# Autodesk Inventor assembly: Chargeur
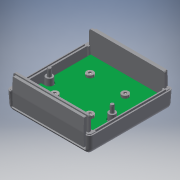
[picture p0: Inventor's stored thumbnail of the model, 180x180]
Saved by Autodesk Inventor 2016 SP1 (Build 200210100, 210)
## iProperties
Created: 2016-04-25
Part Number: Chargeur
Material: Générique
Document SubType Name: Assembly
Designer: dimercur
Sending System: Autodesk Inventor 2016
Preprocessor: unknown
Minimum Resolution: 0.01
Sent Units: Millimeter
Translation Standard: IGES 5.3
Model Creation Time: 2016-02-17
Title: 1593K.iam
Author: MBeerman
## Documents named in this file (8)
- D:\Users\dimercur\Documents\SVN\projets-gei\Dumber 2015\Mecanique\Chargeur\Chargeur.iam
- D:\Users\dimercur\Documents\SVN\projets-gei\Dumber 2015\Mecanique\Chargeur\Hammond\1593K BOTTOM.ipt
- D:\Users\dimercur\Documents\SVN\projets-gei\Dumber 2015\Mecanique\Chargeur\Hammond\1593K Top.ipt
- D:\Users\dimercur\Documents\SVN\projets-gei\Dumber 2015\Mecanique\Chargeur\Hammond\1593K-L-P-Q-X-Y Flat endplate.ipt
- D:\Users\dimercur\Documents\SVN\projets-gei\Dumber 2015\Mecanique\Chargeur\Hammond\1593K-L-P-Q-X-Y Contoured Endplate.ipt
- D:\Users\dimercur\Documents\SVN\projets-gei\Dumber 2015\Mecanique\Chargeur\Hammond\SC549 (screw #4X 3_4'' OH).ipt
- D:\Users\dimercur\Documents\SVN\projets-gei\Dumber 2015\Mecanique\Chargeur\Hammond\1593K PCB.ipt
- D:\Users\dimercur\Documents\Inventor\Content Center Files\R2016\fr-FR\NF E 25-111\NF E 25-111 - M3x6 Classe de qualité 4.8.ipt
## Components (13 placed, 7 different names)
1. 1593K BOTTOM:1
2. 1593K Top:1
3. 1593K-L-P-Q-X-Y Flat endplate:1
4. 1593K-L-P-Q-X-Y Flat endplate:2
5. 1593K-L-P-Q-X-Y Contoured Endplate:1
6. 1593K-L-P-Q-X-Y Contoured Endplate:2
7. SC549 (screw #4X 3_4'' OH):1
8. SC549 (screw #4X 3_4'' OH):2
9. 1593K PCB:1 — Logement:1, Logement:2, Logement:3, Logement:4
10. NF E 25-111 M3x6 Classe de qualité 4.8:1 — Logement:1
11. NF E 25-111 M3x6 Classe de qualité 4.8:2 — Logement:2
12. NF E 25-111 M3x6 Classe de qualité 4.8:3 — Logement:3
13. NF E 25-111 M3x6 Classe de qualité 4.8:4 — Logement:4
## Relationships (4: Insert 4)
- Logement:1 [Insert]: 1593K PCB:1 ↔ NF E 25-111 M3x6 Classe de qualité 4.8:1
- Logement:2 [Insert]: 1593K PCB:1 ↔ NF E 25-111 M3x6 Classe de qualité 4.8:2
- Logement:3 [Insert]: 1593K PCB:1 ↔ NF E 25-111 M3x6 Classe de qualité 4.8:3
- Logement:4 [Insert]: 1593K PCB:1 ↔ NF E 25-111 M3x6 Classe de qualité 4.8:4
